# Autodesk Inventor assembly: Ensamble
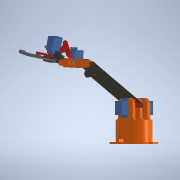
[picture p0: Inventor's stored thumbnail of the model, 180x180]
Saved by Autodesk Inventor 2021 (Build 250183000, 183)
## iProperties
Created: 2021-04-01
Part Number: Ensamble
Document SubType Name: Assembly
Designer: trejo
Author: trejo
## Documents named in this file (16)
- C:\Users\trejo\Documents\Octavo Cuatrimestre\3D Design\homework\Miniproyecto V & VI\Ensamble\Ensamble.iam
- C:\Users\trejo\Documents\Octavo Cuatrimestre\3D Design\homework\Miniproyecto V & VI\elementos\base de la pinza, servo pinza 1 & 2\PIEZA 2.ipt
- C:\Users\trejo\Documents\Octavo Cuatrimestre\3D Design\homework\Miniproyecto V & VI\elementos\eje central del servo, pieza 6 y extensión\servo motor.ipt
- C:\Users\trejo\Documents\Octavo Cuatrimestre\3D Design\homework\Miniproyecto V & VI\elementos\pieza 1, 3 y 4\pieza3parte3.ipt
- C:\Users\trejo\Documents\Octavo Cuatrimestre\3D Design\homework\Miniproyecto V & VI\elementos\pieza 1, 3 y 4\pieza4parte3.ipt
- C:\Users\trejo\Documents\Octavo Cuatrimestre\3D Design\homework\Miniproyecto V & VI\elementos\Eje del servo 1, 2 y pieza 5\eje de servo 1.ipt
- C:\Users\trejo\Documents\Octavo Cuatrimestre\3D Design\homework\Miniproyecto V & VI\elementos\Eje del servo 1, 2 y pieza 5\Pieza 5.ipt
- C:\Users\trejo\Documents\Octavo Cuatrimestre\3D Design\homework\Miniproyecto V & VI\elementos\eje central del servo, pieza 6 y extensión\Extención.ipt
- C:\Users\trejo\Documents\Octavo Cuatrimestre\3D Design\homework\Miniproyecto V & VI\elementos\pieza 1, 3 y 4\basedelapinza1.ipt
- C:\Users\trejo\Documents\Octavo Cuatrimestre\3D Design\homework\Miniproyecto V & VI\elementos\base de la pinza, servo pinza 1 & 2\Base de la pinza 2.ipt
- C:\Users\trejo\Documents\Octavo Cuatrimestre\3D Design\homework\Miniproyecto V & VI\elementos\base de la pinza, servo pinza 1 & 2\Servo pinza 1.ipt
- C:\Users\trejo\Documents\Octavo Cuatrimestre\3D Design\homework\Miniproyecto V & VI\elementos\pieza 1, 3 y 4\base de la pinza.ipt
- C:\Users\trejo\Documents\Octavo Cuatrimestre\3D Design\homework\Miniproyecto V & VI\elementos\base de la pinza, servo pinza 1 & 2\Servo pinza 2 OK.ipt
- C:\Users\trejo\Documents\Octavo Cuatrimestre\3D Design\homework\Miniproyecto V & VI\elementos\eje central del servo, pieza 6 y extensión\Pieza 6.1.ipt
- C:\Users\trejo\Documents\Octavo Cuatrimestre\3D Design\homework\Miniproyecto V & VI\elementos\Eje del servo 1, 2 y pieza 5\eje de servo 2.ipt
- C:\Users\trejo\Documents\Octavo Cuatrimestre\3D Design\homework\Miniproyecto V & VI\elementos\eje central del servo, pieza 6 y extensión\eje central servo.ipt
## Components (22 placed, 15 different names)
1. PIEZA 2:1 — Mate:1, Mate:2, Mate:3, Mate:4, Mate:5, Mate:6, Cylindrical:2, Insert:1, Mate:8, Insert:9, Rotational:20, Rotational:21
2. servo motor:1 — Mate:1, Mate:2, Mate:3, Rotational:2
3. servo motor:2 — Mate:4, Mate:5, Mate:6, Rotational:1
4. pieza4parte3:2 — Mate:8, Mate:9, Mate:11, Insert:5
5. pieza3parte3:1 — Cylindrical:2, Insert:1, Mate:9, Rotational:3
6. eje de servo 1:1 — Rotational:1, Rotational:4
7. eje de servo 1:2 — Rotational:2, Mate:11
8. Pieza 5:1 — Rotational:3, Rotational:8, Insert:6
9. Extención:1 — Rotational:4, Rotational:8
10. basedelapinza1:1 — Insert:3, Insert:4, Rotational:16, Rotational:17, Rotational:18, Insert:6
11. Base de la pinza 2:1 — Insert:3, Insert:4, Mate:13, Mate:14, Mate:15, Insert:8
12. servo motor:3 — Mate:13, Mate:14, Mate:15, Rotational:15
13. eje de servo 1:3 — Rotational:15, Mate:16
14. base de la pinza:1 — Rotational:21, Insert:10, Mate:20
15. Servo pinza 2 OK:1 — Rotational:16, Mate:16
16. Servo pinza 1:1 — Rotational:17
17. Pieza 6.1:1 — Insert:5, Rotational:18, Insert:7, Mate:17, Mate:18
18. servo motor:4 — Insert:7, Mate:17, Mate:18, Rotational:19
19. eje de servo 2:1 — Insert:8, Mate:19
20. eje de servo 1:4 — Rotational:19, Mate:19
21. servo motor:5 — Insert:10, Mate:20
22. eje central servo:1 — Insert:9, Rotational:20
## Relationships (39: Mate 17, RevoluteJoint 12, Insert 9, CylindricalJoint 1)
- Mate:1: PIEZA 2:1 ↔ servo motor:1
- Mate:2: PIEZA 2:1 ↔ servo motor:1
- Mate:3: PIEZA 2:1 ↔ servo motor:1
- Mate:4: PIEZA 2:1 ↔ servo motor:2
- Mate:5: PIEZA 2:1 ↔ servo motor:2
- Mate:6: PIEZA 2:1 ↔ servo motor:2
- Cylindrical:2: PIEZA 2:1 ↔ pieza3parte3:1
- Insert:1: PIEZA 2:1 ↔ pieza3parte3:1
- Mate:8: PIEZA 2:1 ↔ pieza4parte3:2
- Mate:9: pieza4parte3:2 ↔ pieza3parte3:1
- Rotational:1 [RevoluteJoint]: servo motor:2 ↔ eje de servo 1:1
- Rotational:2 [RevoluteJoint]: servo motor:1 ↔ eje de servo 1:2
- Mate:11: pieza4parte3:2 ↔ eje de servo 1:2
- Rotational:3 [RevoluteJoint]: pieza3parte3:1 ↔ Pieza 5:1
- Rotational:4 [RevoluteJoint]: eje de servo 1:1 ↔ Extención:1
- Insert:3: basedelapinza1:1 ↔ Base de la pinza 2:1
- Insert:4: basedelapinza1:1 ↔ Base de la pinza 2:1
- Rotational:8 [RevoluteJoint]: Pieza 5:1 ↔ Extención:1
- Mate:13: Base de la pinza 2:1 ↔ servo motor:3
- Mate:14: Base de la pinza 2:1 ↔ servo motor:3
- Mate:15: Base de la pinza 2:1 ↔ servo motor:3
- Rotational:15 [RevoluteJoint]: servo motor:3 ↔ eje de servo 1:3
- Rotational:16 [RevoluteJoint]: basedelapinza1:1 ↔ Servo pinza 2 OK:1
- Mate:16: eje de servo 1:3 ↔ Servo pinza 2 OK:1
- Rotational:17 [RevoluteJoint]: basedelapinza1:1 ↔ Servo pinza 1:1
- Insert:5: pieza4parte3:2 ↔ Pieza 6.1:1
- Rotational:18 [RevoluteJoint]: basedelapinza1:1 ↔ Pieza 6.1:1
- Insert:6: Pieza 5:1 ↔ basedelapinza1:1
- Insert:7: Pieza 6.1:1 ↔ servo motor:4
- Mate:17: Pieza 6.1:1 ↔ servo motor:4
- Mate:18: Pieza 6.1:1 ↔ servo motor:4
- Insert:8: Base de la pinza 2:1 ↔ eje de servo 2:1
- Rotational:19 [RevoluteJoint]: servo motor:4 ↔ eje de servo 1:4
- Mate:19: eje de servo 2:1 ↔ eje de servo 1:4
- Insert:9: PIEZA 2:1 ↔ eje central servo:1
- Rotational:20 [RevoluteJoint]: PIEZA 2:1 ↔ eje central servo:1
- Rotational:21 [RevoluteJoint]: PIEZA 2:1 ↔ base de la pinza:1
- Insert:10: base de la pinza:1 ↔ servo motor:5
- Mate:20: base de la pinza:1 ↔ servo motor:5
